# Autodesk Inventor assembly: bottom_roller
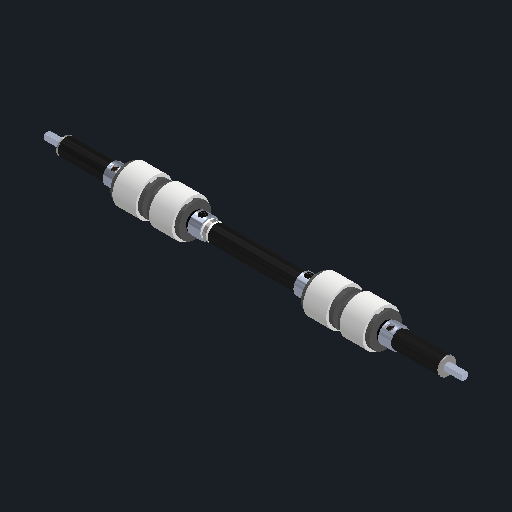
[picture p0: Inventor's stored thumbnail of the model, 512x512]
Saved by Autodesk Inventor 2025 (Build 290162000, 162)
## iProperties
Created: 2024-08-18
Part Number: bottom_roller
Document SubType Name: Assembly
Designer: averey
Author: averey
## Documents named in this file (17)
- D:\vex_robotics_high_stakes\hardware\cad\bots\ENIGMA\intake\first_stage\bottom_roller.iam
- D:\vex_robotics_high_stakes\hardware\cad\_quick_assemblies\0.8125_flex_wheel_w_versahex.iam
- D:\vex_robotics_high_stakes\hardware\cad\VEX-CAD-Inventor\Motion\Shaft LS\Shaft Collar ipts\Shaft Collar Set Screw.ipt
- D:\vex_robotics_high_stakes\hardware\cad\VEX-CAD-Inventor\Motion\Spacers\Spacer Nylon .375 OD\NSpacer .375 OD x .500.ipt
- C:\Users\avere\vex_robotics_high_stakes\hardware\cad\VEX-CAD-Inventor\Motion\Spacers\Spacer Nylon .375 OD.ipt
- D:\vex_robotics_high_stakes\hardware\cad\VEX-CAD-Inventor\Motion\Spacers\Spacer Nylon .375 OD\NSpacer .375 OD x .375.ipt
- D:\vex_robotics_high_stakes\hardware\cad\VEX-CAD-Inventor\Motion\Spacers\Washer Teflon\TWasher .375 OD x .04000.ipt
- C:\Users\avere\vex_robotics_high_stakes\hardware\cad\VEX-CAD-Inventor\Motion\Spacers\Washer Teflon.ipt
- D:\vex_robotics_high_stakes\hardware\cad\VEX-CAD-Inventor\Motion\Spacers\Washer Steel\SWasher .375 OD x .015625.ipt
- C:\Users\avere\vex_robotics_high_stakes\hardware\cad\VEX-CAD-Inventor\Motion\Spacers\Washer Steel.ipt
- D:\vex_robotics_high_stakes\hardware\cad\VEX-CAD-Inventor\Motion\Spacers\Spacer Nylon .375 OD\NSpacer .375 OD x .250.ipt
- D:\vex_robotics_high_stakes\hardware\cad\VEX-CAD-Inventor\Motion\Spacers\Washer Steel\SWasher .375 OD x .031250.ipt
- D:\vex_robotics_high_stakes\hardware\cad\VEX-CAD-Inventor\Motion\Spacers\Washer Steel\SWasher .375 OD x .062500.ipt
- C:\Users\avere\vex_robotics_high_stakes\hardware\cad\VEX-CAD-Inventor\Motion\Shaft LS\Shaft LS.ipt
- D:\vex_robotics_high_stakes\hardware\cad\VEX-CAD-Inventor\Motion\Shaft LS\Shaft LS\Shaft LS 8.0.ipt
- D:\vex_robotics_high_stakes\hardware\cad\VEX-CAD-Inventor\Motion\Shaft LS\Shaft LS\Shaft LS 9.0.ipt
- D:\vex_robotics_high_stakes\hardware\cad\VEX-CAD-Inventor\Motion\Shaft LS\Shaft Collar ipts\Shaft Collar No Screw.ipt
## Components (26 placed, 12 different names)
1. 0.8125_flex_wheel_w_versahex:1 [sub-assembly] — Insert:17, Insert:27
2. 0.8125_flex_wheel_w_versahex:2 [sub-assembly]
3. 0.8125_flex_wheel_w_versahex:3 [sub-assembly]
4. 0.8125_flex_wheel_w_versahex:4 [sub-assembly] — Insert:14, Insert:28
5. Shaft Collar Set Screw:1
6. Shaft Collar Set Screw:2 — Insert:20
7. NSpacer .375 OD x .500:1
8. NSpacer .375 OD x .500:2
9. NSpacer .375 OD x .500:3
10. NSpacer .375 OD x .375:4
11. TWasher .375 OD x .04000:1
12. SWasher .375 OD x .015625:1 — Insert:19
13. NSpacer .375 OD x .250:5 — Insert:13, Insert:14
14. NSpacer .375 OD x .500:6 — Insert:13, Insert:25
15. SWasher .375 OD x .031250:2 — Insert:26
16. NSpacer .375 OD x .250:7 — Insert:17
17. NSpacer .375 OD x .500:8 — Insert:23
18. SWasher .375 OD x .031250:3 — Insert:24
19. SWasher .375 OD x .062500:4 — Insert:19
20. TWasher .375 OD x .04000:2 — Insert:20
21. Shaft LS 8.0:1 — Insert:22
22. Shaft LS 9.0:2 — Insert:22
23. NSpacer .375 OD x .500:9 — Insert:23, Insert:24
24. NSpacer .375 OD x .500:10 — Insert:25, Insert:26
25. Shaft Collar No Screw:1 — Insert:27
26. Shaft Collar No Screw:2 — Insert:28
## Relationships (25: Insert 24, Mate 1)
- [Insert]: 0.8125_flex_wheel_w_versahex:1 ↔ 0.8125_flex_wheel_w_versahex:2
- [Mate]: 0.8125_flex_wheel_w_versahex:2 ↔ 0.8125_flex_wheel_w_versahex:3
- [Insert]: 0.8125_flex_wheel_w_versahex:3 ↔ 0.8125_flex_wheel_w_versahex:4
- [Insert]: TWasher .375 OD x .04000:1 ↔ SWasher .375 OD x .015625:1
- [Insert]: NSpacer .375 OD x .500:2 ↔ TWasher .375 OD x .04000:1
- [Insert]: NSpacer .375 OD x .500:1 ↔ NSpacer .375 OD x .375:4
- [Insert]: NSpacer .375 OD x .500:1 ↔ NSpacer .375 OD x .500:3
- [Insert]: NSpacer .375 OD x .500:2 ↔ NSpacer .375 OD x .500:3
- [Insert]: 0.8125_flex_wheel_w_versahex:2 ↔ Shaft Collar Set Screw:2
- [Insert]: Shaft Collar Set Screw:1 ↔ NSpacer .375 OD x .375:4
- [Insert] (0.0424 mm): 0.8125_flex_wheel_w_versahex:3 ↔ Shaft Collar Set Screw:1
- Insert:13: NSpacer .375 OD x .250:5 ↔ NSpacer .375 OD x .500:6
- Insert:14: 0.8125_flex_wheel_w_versahex:4 ↔ NSpacer .375 OD x .250:5
- [Insert]: NSpacer .375 OD x .250:7 ↔ NSpacer .375 OD x .500:8
- Insert:17: 0.8125_flex_wheel_w_versahex:1 ↔ NSpacer .375 OD x .250:7
- [Insert]: SWasher .375 OD x .062500:4 ↔ TWasher .375 OD x .04000:2
- Insert:19: SWasher .375 OD x .015625:1 ↔ SWasher .375 OD x .062500:4
- Insert:20: Shaft Collar Set Screw:2 ↔ TWasher .375 OD x .04000:2
- Insert:22 (-12.7 mm): Shaft LS 8.0:1 ↔ Shaft LS 9.0:2
- Insert:23: NSpacer .375 OD x .500:8 ↔ NSpacer .375 OD x .500:9
- Insert:24: SWasher .375 OD x .031250:3 ↔ NSpacer .375 OD x .500:9
- Insert:25: NSpacer .375 OD x .500:6 ↔ NSpacer .375 OD x .500:10
- Insert:26: SWasher .375 OD x .031250:2 ↔ NSpacer .375 OD x .500:10
- Insert:27 (0.0794 mm): 0.8125_flex_wheel_w_versahex:1 ↔ Shaft Collar No Screw:1
- Insert:28 (0.0794 mm): 0.8125_flex_wheel_w_versahex:4 ↔ Shaft Collar No Screw:2
## Named parameters: d0_d9 = 0 mm, d1_d10 = 0 mm, d17_d14 = 0 mm
